# Autodesk Inventor assembly: -ZPanel
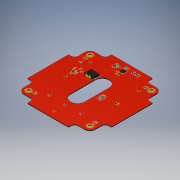
[picture p0: Inventor's stored thumbnail of the model, 180x180]
Saved by Autodesk Inventor 2018 (Build 220112000, 112)
## iProperties
Created: 2018-11-03
Part Number: -ZPanel
Document SubType Name: Assembly
Designer: Bradley
Author: Bradley
## Documents named in this file (16)
- C:\Users\Bradley\Documents\GitHub\CougSat1-Hardware\CougSat1-RadioBoard\CADModel\Native\-ZPanel.iam
- C:\Users\Bradley\Documents\GitHub\CougSat1-Hardware\CougSat1-RadioBoard\CADModel\Native\-ZPanel_PCB.ipt
- C:\Users\Bradley\Documents\GitHub\Resources\SupplierDocuments\04 - Connectors SMT\04-0001\04-0001.iam
- C:\Users\Bradley\Documents\GitHub\Resources\SupplierDocuments\21 - Resistor 1608\21-0000\21-0000.ipt
- C:\Users\Bradley\Documents\GitHub\Resources\SupplierDocuments\36 - Ferrite\36-152A\36-152A.ipt
- C:\Users\Bradley\Documents\GitHub\Resources\SupplierDocuments\11 - Capacitor Ceramic 1608\11-105A\11-105A.ipt
- C:\Users\Bradley\Documents\GitHub\Resources\SupplierDocuments\21 - Resistor 1608\21-1001\21-1001.ipt
- C:\Users\Bradley\Documents\GitHub\Resources\SupplierDocuments\16 - Capacitor Tantalum SMT\16-475A\16-475A.ipt
- C:\Users\Bradley\Documents\GitHub\Resources\SupplierDocuments\11 - Capacitor Ceramic 1608\11-106A\11-106A.ipt
- C:\Users\Bradley\Documents\GitHub\Resources\SupplierDocuments\26 - Resistor Misc\26-0000\26-0000.ipt
- C:\Users\Bradley\Documents\GitHub\Resources\SupplierDocuments\26 - Resistor Misc\26-0008\26-0008.ipt
- C:\Users\Bradley\Documents\GitHub\Resources\SupplierDocuments\11 - Capacitor Ceramic 1608\11-104A\11-104A.ipt
- C:\Users\Bradley\Documents\GitHub\Resources\SupplierDocuments\21 - Resistor 1608\21-1500\21-1500.ipt
- C:\Users\Bradley\Documents\GitHub\Resources\SupplierDocuments\27 - Conversion IC\27-0003\27-0003.ipt
- C:\Users\Bradley\Documents\GitHub\Resources\SupplierDocuments\08 - Amplifier (excluding RF)\08-0002\08-0002.ipt
- C:\Users\Bradley\Documents\GitHub\Resources\SupplierDocuments\66 - Sensor\66-0003\66-0003.ipt
## Components (34 placed, 15 different names)
1. 66-0003:1 — Mate:82, Mate:83, Flush:16
2. 08-0002:1 — Mate:80, Flush:15, Mate:81
3. 27-0003:1 — Mate:78, Mate:79, Flush:14
4. 21-1500:1 — Mate:75, Mate:76, Mate:77
5. 11-104A:8 — Mate:62, Mate:73, Mate:74
6. 11-104A:7 — Mate:61, Mate:71, Mate:72
7. 11-104A:6 — Mate:60, Mate:70, Flush:13
8. 11-104A:5 — Mate:59, Mate:69, Flush:12
9. 11-104A:4 — Mate:58, Mate:68, Flush:11
10. 11-104A:3 — Mate:57, Mate:67, Flush:10
11. 11-104A:2 — Mate:56, Mate:65, Mate:66
12. 11-104A:1 — Mate:55, Mate:63, Mate:64
13. 26-0008:7 — Mate:44, Mate:54, Flush:9
14. 26-0008:6 — Mate:43, Mate:53, Flush:8
15. 26-0008:5 — Mate:42, Mate:51, Mate:52
16. 26-0008:4 — Mate:41, Mate:49, Mate:50
17. 26-0008:3 — Mate:40, Mate:47, Mate:48
18. 26-0008:2 — Mate:39, Mate:46, Flush:7
19. 26-0008:1 — Mate:38, Mate:45, Flush:6
20. 26-0000:2 — Mate:33, Mate:36, Mate:37
21. 26-0000:1 — Mate:32, Mate:34, Mate:35
22. 11-106A:1 — Mate:30, Mate:31, Flush:5
23. 16-475A:1 — Mate:27, Mate:28, Mate:29
24. 21-1001:1 — Mate:24, Mate:25, Mate:26
25. 11-105A:1 — Mate:21, Mate:22, Mate:23
26. 36-152A:1 — Mate:19, Mate:20, Flush:4
27. 21-0000:6 — Mate:6, Mate:17, Mate:18
28. 21-0000:5 — Mate:7, Mate:16, Flush:3
29. 21-0000:4 — Mate:8, Mate:14, Mate:15
30. 21-0000:3 — Mate:9, Mate:12, Mate:13
31. 21-0000:2 — Mate:5, Mate:11, Flush:2
32. 21-0000:1 — Mate:4, Mate:10, Flush:1
33. 04-0001:1 [sub-assembly] — Mate:1, Mate:2, Mate:3
34. -ZPanel_PCB:1 — Mate:1, Mate:4, Mate:5, Mate:6, Mate:7, Mate:8, Mate:9, Mate:19, Mate:21, Mate:24, Mate:27, Mate:30, Mate:32, Mate:33, Mate:38, Mate:39, Mate:40, Mate:41, Mate:42, Mate:43, Mate:44, Mate:55, Mate:56, Mate:57, Mate:58, Mate:59, Mate:60, Mate:61, Mate:62, Mate:75, Mate:78, Mate:80, Mate:82
## Relationships (99: Mate 83, Flush 16)
- Mate:1: 04-0001:1 ↔ -ZPanel_PCB:1
- Mate:2 (-14 mm): 04-0001:1
- Mate:3 (20 mm): 04-0001:1
- Mate:4: 21-0000:1 ↔ -ZPanel_PCB:1
- Mate:5: 21-0000:2 ↔ -ZPanel_PCB:1
- Mate:6: 21-0000:6 ↔ -ZPanel_PCB:1
- Mate:7: 21-0000:5 ↔ -ZPanel_PCB:1
- Mate:8: 21-0000:4 ↔ -ZPanel_PCB:1
- Mate:9: 21-0000:3 ↔ -ZPanel_PCB:1
- Mate:10 (42 mm): 21-0000:1
- Flush:1 (1 mm): 21-0000:1
- Mate:11 (-34.25 mm): 21-0000:2
- Flush:2 (29.5 mm): 21-0000:2
- Mate:12 (-35 mm): 21-0000:3
- Mate:13 (30.25 mm): 21-0000:3
- Mate:14 (35 mm): 21-0000:4
- Mate:15 (-29.5 mm): 21-0000:4
- Mate:16 (34.25 mm): 21-0000:5
- Flush:3 (-30 mm): 21-0000:5
- Mate:17 (-33.5 mm): 21-0000:6
- Mate:18 (22.5 mm): 21-0000:6
- Mate:19: 36-152A:1 ↔ -ZPanel_PCB:1
- Mate:20 (-23.5 mm): 36-152A:1
- Flush:4 (-14.5 mm): 36-152A:1
- Mate:21: 11-105A:1 ↔ -ZPanel_PCB:1
- Mate:22 (42 mm): 11-105A:1
- Mate:23 (0.75 mm): 11-105A:1
- Mate:24: 21-1001:1 ↔ -ZPanel_PCB:1
- Mate:25 (-1 mm): 21-1001:1
- Mate:26 (31.5 mm): 21-1001:1
- Mate:27: 16-475A:1 ↔ -ZPanel_PCB:1
- Mate:28 (-27.25 mm): 16-475A:1
- Mate:29 (9.5 mm): 16-475A:1
- Mate:30: 11-106A:1 ↔ -ZPanel_PCB:1
- Mate:31 (-10.25 mm): 11-106A:1
- Flush:5 (-41.5 mm): 11-106A:1
- Mate:32: 26-0000:1 ↔ -ZPanel_PCB:1
- Mate:33: 26-0000:2 ↔ -ZPanel_PCB:1
- Mate:34 (7.93 mm): 26-0000:1
- Mate:35 (41.81 mm): 26-0000:1
- Mate:36 (12.6 mm): 26-0000:2
- Mate:37 (41.81 mm): 26-0000:2
- Mate:38: 26-0008:1 ↔ -ZPanel_PCB:1
- Mate:39: 26-0008:2 ↔ -ZPanel_PCB:1
- Mate:40: 26-0008:3 ↔ -ZPanel_PCB:1
- Mate:41: 26-0008:4 ↔ -ZPanel_PCB:1
- Mate:42: 26-0008:5 ↔ -ZPanel_PCB:1
- Mate:43: 26-0008:6 ↔ -ZPanel_PCB:1
- Mate:44: 26-0008:7 ↔ -ZPanel_PCB:1
- Mate:45 (-28 mm): 26-0008:1
- Flush:6 (-28 mm): 26-0008:1
- Mate:46 (-28 mm): 26-0008:2
- Flush:7: 26-0008:2
- Mate:47 (-28 mm): 26-0008:3
- Mate:48 (-18 mm): 26-0008:3
- Mate:49 (-28 mm): 26-0008:4
- Mate:50: 26-0008:4
- Mate:51 (-28 mm): 26-0008:5
- Mate:52 (18 mm): 26-0008:5
- Mate:53 (28 mm): 26-0008:6
- Flush:8 (-1.5 mm): 26-0008:6
- Mate:54 (28 mm): 26-0008:7
- Flush:9 (-28 mm): 26-0008:7
- Mate:55: 11-104A:1 ↔ -ZPanel_PCB:1
- Mate:56: 11-104A:2 ↔ -ZPanel_PCB:1
- Mate:57: 11-104A:3 ↔ -ZPanel_PCB:1
- Mate:58: 11-104A:4 ↔ -ZPanel_PCB:1
- Mate:59: 11-104A:5 ↔ -ZPanel_PCB:1
- Mate:60: 11-104A:6 ↔ -ZPanel_PCB:1
- Mate:61: 11-104A:7 ↔ -ZPanel_PCB:1
- Mate:62: 11-104A:8 ↔ -ZPanel_PCB:1
- Mate:63 (-34.25 mm): 11-104A:1
- Mate:64 (-27.75 mm): 11-104A:1
- Mate:65 (42 mm): 11-104A:2
- Mate:66 (-2.75 mm): 11-104A:2
- Mate:67 (-2.5 mm): 11-104A:3
- Flush:10 (-33.75 mm): 11-104A:3
- Mate:68 (-28 mm): 11-104A:4
- Flush:11 (-6 mm): 11-104A:4
- Mate:69 (-35 mm): 11-104A:5
- Flush:12 (-28.5 mm): 11-104A:5
- Mate:70 (35 mm): 11-104A:6
- Flush:13 (27.75 mm): 11-104A:6
- Mate:71 (34.25 mm): 11-104A:7
- Mate:72 (28.25 mm): 11-104A:7
- Mate:73 (39.5 mm): 11-104A:8
- Mate:74 (-7 mm): 11-104A:8
- Mate:75: 21-1500:1 ↔ -ZPanel_PCB:1
- Mate:76 (28 mm): 21-1500:1
- Mate:77 (3.5 mm): 21-1500:1
- Mate:78: 27-0003:1 ↔ -ZPanel_PCB:1
- Mate:79 (0.25 mm): 27-0003:1
- Flush:14 (-37.5 mm): 27-0003:1
- Mate:80: 08-0002:1 ↔ -ZPanel_PCB:1
- Flush:15 (-9.9 mm): 08-0002:1
- Mate:81 (37.98 mm): 08-0002:1
- Mate:82: 66-0003:1 ↔ -ZPanel_PCB:1
- Mate:83: 66-0003:1
- Flush:16 (-14 mm): 66-0003:1
